# Autodesk Inventor assembly: SideShaftB
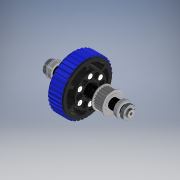
[picture p0: Inventor's stored thumbnail of the model, 180x180]
Saved by Autodesk Inventor 2018 (Build 220112000, 112)
## iProperties
Created: 2017-09-03
Part Number: SideShaftB
Document SubType Name: Assembly
Designer: snipe
Author: snipe
## Documents named in this file (9)
- E:\Clark\Assets\SideShaftB.iam
- E:\Clark\Assets\ThunderHex_SideShaft.ipt
- E:\Clark\Assets\FlangedThunderHexBearing.ipt
- E:\Clark\Assets\ShaftCollar.ipt
- E:\Clark\Assets\0.5inSpacer.ipt
- E:\Clark\Assets\0.25inSpacer.ipt
- E:\Clark\Assets\0.125inSpacer.ipt
- E:\Clark\Assets\PlactionWheelwithHubnoBearing.iam
- E:\Clark\Assets\24tPulley15mm.ipt
## Components (17 placed, 8 different names)
1. ThunderHex_SideShaft:1 — Flush:1, Mate:1, Mate:2, Mate:4, Mate:5, Mate:7, Mate:9, Mate:10, Mate:12, Mate:13, Mate:15, Mate:16, Mate:24, Mate:25, Mate:27, Mate:28, Mate:30, Mate:32, Mate:33, Mate:35, Mate:36, Mate:40, Mate:41, Mate:43, Mate:44, Mate:45, Mate:46, Mate:47, Mate:48, Mate:50, Mate:51
2. FlangedThunderHexBearing:1 — Mate:29, Mate:30, Mate:31
3. FlangedThunderHexBearing:2 — Mate:6, Mate:7, Mate:8
4. ShaftCollar:1 — Flush:1, Mate:1, Mate:2, Mate:3
5. ShaftCollar:2 — Mate:34, Mate:35, Mate:36
6. 0.5inSpacer:1 — Mate:8, Mate:9, Mate:10, Mate:11
7. 0.5inSpacer:2 — Mate:24, Mate:25, Mate:26
8. 0.25inSpacer:1 — Mate:11, Mate:12, Mate:13, Mate:14
9. 0.125inSpacer:1 — Mate:26, Mate:27, Mate:28, Mate:29
10. 0.125inSpacer:2 — Mate:31, Mate:32, Mate:33, Mate:34
11. 0.125inSpacer:3 — Mate:3, Mate:4, Mate:5, Mate:6
12. PlactionWheelwithHubnoBearing:1 [sub-assembly] — Mate:14, Mate:15, Mate:16, Mate:42
13. 0.5inSpacer:3 — Mate:37, Mate:40, Mate:41, Mate:42
14. 0.5inSpacer:4 — Mate:37, Mate:38, Mate:43, Mate:46
15. 0.5inSpacer:5 — Mate:38, Mate:39, Mate:44, Mate:47
16. 0.25inSpacer:2 — Mate:39, Mate:45, Mate:48, Mate:49
17. 24tPulley15mm:1 — Mate:49, Mate:50, Mate:51
## Relationships (45: Mate 44, Flush 1)
- Flush:1: ThunderHex_SideShaft:1 ↔ ShaftCollar:1
- Mate:1: ThunderHex_SideShaft:1 ↔ ShaftCollar:1
- Mate:2: ThunderHex_SideShaft:1 ↔ ShaftCollar:1
- Mate:3: ShaftCollar:1 ↔ 0.125inSpacer:3
- Mate:4: ThunderHex_SideShaft:1 ↔ 0.125inSpacer:3
- Mate:5: ThunderHex_SideShaft:1 ↔ 0.125inSpacer:3
- Mate:6: FlangedThunderHexBearing:2 ↔ 0.125inSpacer:3
- Mate:7: ThunderHex_SideShaft:1 ↔ FlangedThunderHexBearing:2
- Mate:8: FlangedThunderHexBearing:2 ↔ 0.5inSpacer:1
- Mate:9: ThunderHex_SideShaft:1 ↔ 0.5inSpacer:1
- Mate:10: ThunderHex_SideShaft:1 ↔ 0.5inSpacer:1
- Mate:11: 0.5inSpacer:1 ↔ 0.25inSpacer:1
- Mate:12: ThunderHex_SideShaft:1 ↔ 0.25inSpacer:1
- Mate:13: ThunderHex_SideShaft:1 ↔ 0.25inSpacer:1
- Mate:14: 0.25inSpacer:1 ↔ PlactionWheelwithHubnoBearing:1
- Mate:15: ThunderHex_SideShaft:1 ↔ PlactionWheelwithHubnoBearing:1
- Mate:16: ThunderHex_SideShaft:1 ↔ PlactionWheelwithHubnoBearing:1
- Mate:24: ThunderHex_SideShaft:1 ↔ 0.5inSpacer:2
- Mate:25: ThunderHex_SideShaft:1 ↔ 0.5inSpacer:2
- Mate:26: 0.5inSpacer:2 ↔ 0.125inSpacer:1
- Mate:27: ThunderHex_SideShaft:1 ↔ 0.125inSpacer:1
- Mate:28: ThunderHex_SideShaft:1 ↔ 0.125inSpacer:1
- Mate:29: FlangedThunderHexBearing:1 ↔ 0.125inSpacer:1
- Mate:30: ThunderHex_SideShaft:1 ↔ FlangedThunderHexBearing:1
- Mate:31: FlangedThunderHexBearing:1 ↔ 0.125inSpacer:2
- Mate:32: ThunderHex_SideShaft:1 ↔ 0.125inSpacer:2
- Mate:33: ThunderHex_SideShaft:1 ↔ 0.125inSpacer:2
- Mate:34: ShaftCollar:2 ↔ 0.125inSpacer:2
- Mate:35: ThunderHex_SideShaft:1 ↔ ShaftCollar:2
- Mate:36: ThunderHex_SideShaft:1 ↔ ShaftCollar:2
- Mate:37: 0.5inSpacer:3 ↔ 0.5inSpacer:4
- Mate:38: 0.5inSpacer:4 ↔ 0.5inSpacer:5
- Mate:39: 0.5inSpacer:5 ↔ 0.25inSpacer:2
- Mate:40: ThunderHex_SideShaft:1 ↔ 0.5inSpacer:3
- Mate:41: ThunderHex_SideShaft:1 ↔ 0.5inSpacer:3
- Mate:42: PlactionWheelwithHubnoBearing:1 ↔ 0.5inSpacer:3
- Mate:43: ThunderHex_SideShaft:1 ↔ 0.5inSpacer:4
- Mate:44: ThunderHex_SideShaft:1 ↔ 0.5inSpacer:5
- Mate:45: ThunderHex_SideShaft:1 ↔ 0.25inSpacer:2
- Mate:46: ThunderHex_SideShaft:1 ↔ 0.5inSpacer:4
- Mate:47: ThunderHex_SideShaft:1 ↔ 0.5inSpacer:5
- Mate:48: ThunderHex_SideShaft:1 ↔ 0.25inSpacer:2
- Mate:49: 0.25inSpacer:2 ↔ 24tPulley15mm:1
- Mate:50: ThunderHex_SideShaft:1 ↔ 24tPulley15mm:1
- Mate:51: ThunderHex_SideShaft:1 ↔ 24tPulley15mm:1
